# Autodesk Inventor assembly: Tire
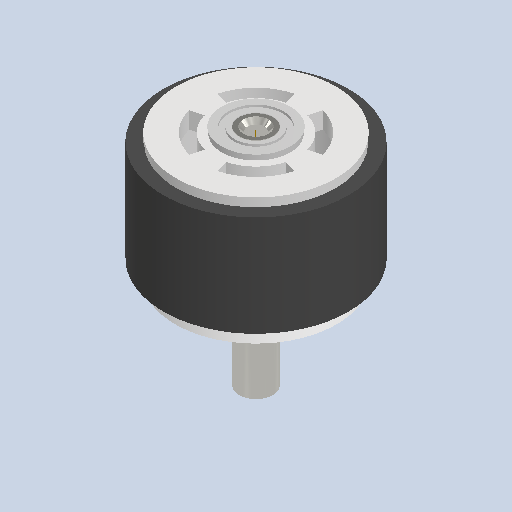
[picture p0: Inventor's stored thumbnail of the model, 512x512]
Saved by Autodesk Inventor 2022 (Build 260153000, 153)
## iProperties
Created: 2021-09-23
Part Number: Tire
Document SubType Name: Assembly
Designer: shiok
Mass: 6.39582 g
Surface Area: 59.289 cm^2
Volume: 3.61915 cm^3
Density: 1.76722 g/cm^3
Author: shiok
## Documents named in this file (7)
- C:\Users\Yazawa\Documents\GitHub\murakumo\inventor\Tire.iam
- C:\Users\Yazawa\Documents\GitHub\murakumo\inventor\wheel.ipt
- C:\Users\Yazawa\Documents\GitHub\murakumo\inventor\wheelcap.ipt
- C:\Users\Yazawa\Documents\GitHub\murakumo\inventor\Tire.ipt
- C:\Users\Yazawa\Documents\GitHub\murakumo\inventor\spergear.ipt
- C:\Users\Yazawa\Documents\GitHub\murakumo\inventor\FL674ZZ.ipt
- C:\Users\Yazawa\Documents\GitHub\murakumo\inventor\shaft.ipt
## Components (8 placed, 6 different names)
1. wheel:1 — 挿入:1, 挿入:2, メイト:1, 挿入:3, メイト:4, メイト:5
2. wheelcap:1 — 挿入:1, メイト:6, メイト:7
3. Tire:1 — 挿入:2
4. spergear:1 — メイト:1, 挿入:3, メイト:2, メイト:3
5. FL674ZZ:1 — メイト:2, メイト:3
6. FL674ZZ:2 — メイト:4, メイト:5
7. FL674ZZ:3 — メイト:6, メイト:7, フラッシュ:1, メイト:8, フラッシュ:2, フラッシュ:3
8. shaft:1 — フラッシュ:1, メイト:8, フラッシュ:2, フラッシュ:3
## Relationships (14: Mate 8, Insert 3, Flush 3)
- 挿入:1 [Insert]: wheel:1 ↔ wheelcap:1
- 挿入:2 [Insert]: wheel:1 ↔ Tire:1
- メイト:1 [Mate]: wheel:1 ↔ spergear:1
- 挿入:3 [Insert]: wheel:1 ↔ spergear:1
- メイト:2 [Mate]: spergear:1 ↔ FL674ZZ:1
- メイト:3 [Mate]: spergear:1 ↔ FL674ZZ:1
- メイト:4 [Mate]: wheel:1 ↔ FL674ZZ:2
- メイト:5 [Mate]: wheel:1 ↔ FL674ZZ:2
- メイト:6 [Mate]: wheelcap:1 ↔ FL674ZZ:3
- メイト:7 [Mate]: wheelcap:1 ↔ FL674ZZ:3
- フラッシュ:1 [Flush]: FL674ZZ:3 ↔ shaft:1
- メイト:8 [Mate]: FL674ZZ:3 ↔ shaft:1
- フラッシュ:2 [Flush]: FL674ZZ:3 ↔ shaft:1
- フラッシュ:3 [Flush]: FL674ZZ:3 ↔ shaft:1
